# Autodesk Inventor assembly: board_box
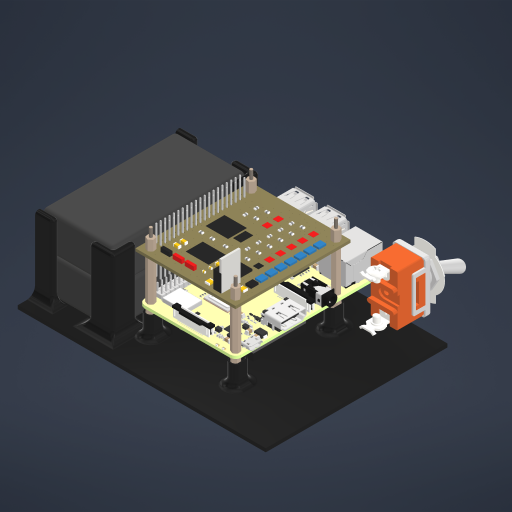
[picture p0: Inventor's stored thumbnail of the model, 512x512]
Saved by Autodesk Inventor 2023 (Build 270158030, 158C)
## iProperties
Created: 2022-07-10
Part Number: board_box
Document SubType Name: Assembly
Designer: Norbert Ligas
Author: Norbert Ligas
## Documents named in this file (10)
- C:\Users\norbe\Repozytoria\NormalMapScanner\3D_modeling\construction\parts\board_box.iam
- C:\Users\norbe\Repozytoria\NormalMapScanner\3D_modeling\power_supply_pcb\power_supply.iam
- C:\Users\norbe\Repozytoria\NormalMapScanner\3D_modeling\construction\parts\board_box\spacer25.ipt
- C:\Users\norbe\Repozytoria\NormalMapScanner\3D_modeling\construction\parts\external_parts\raspberry_pi_3_b_plus\raspberry_pi_3_b_plus.iam
- C:\Users\norbe\Repozytoria\NormalMapScanner\3D_modeling\construction\parts\board_box\RaspberryCameraV2InCase.iam
- C:\Users\norbe\Repozytoria\NormalMapScanner\3D_modeling\construction\parts\board_box\board_box_bottom.ipt
- C:\Users\norbe\Repozytoria\NormalMapScanner\3D_modeling\construction\parts\board_box\RaspberryCameraV2Case.ipt
- C:\Users\norbe\Repozytoria\NormalMapScanner\3D_modeling\construction\parts\board_box\accumulators_case.ipt
- C:\Users\norbe\Repozytoria\NormalMapScanner\3D_modeling\construction\parts\board_box\spacer6.ipt
- C:\Users\norbe\Repozytoria\NormalMapScanner\3D_modeling\construction\parts\board_box\Switch\Switch.iam
## Components (19 placed, 8 different names)
1. raspberry_pi_3_b_plus:2 [sub-assembly] — Mate:20, Mate:22, Mate:34, Mate:35, Mate:36, Mate:42, Mate:46, Mate:47, Mate:54, Mate:55, Mate:56, Mate:58, Mate:60, Mate:62
2. power_supply:1 [sub-assembly] — Mate:41, Mate:44, Mate:45, Mate:63, Mate:65, Mate:66, Mate:67, Mate:68, Mate:69, Mate:71, Mate:73, Mate:75
3. spacer25:1 — Mate:20, Mate:38, Mate:54, Mate:59, Mate:60, Mate:67
4. spacer25:2 — Mate:61, Mate:62, Mate:69, Mate:70
5. spacer25:3 — Mate:22, Mate:63, Mate:65, Mate:66, Mate:72
6. spacer25:4 — Mate:57, Mate:58, Mate:68, Mate:74
7. RaspberryCameraV2InCase:1 [sub-assembly] — Mate:51, Mate:52, Flush:5, Flush:6, Mate:81, Mate:82, Mate:83
8. board_box_bottom:1 — Mate:51, Mate:76, Mate:77, Mate:78, Mate:79, Mate:80, Flush:6, Mate:82, Mate:83, Flush:8, Mate:84, Mate:85, Mate:86
9. accumulators_case:1 — Mate:28, Flush:3, Flush:4, Mate:84, Mate:85, Mate:86
10. accumulators_case:2 — Mate:28, Flush:3, Flush:4
11. spacer6:1 — Mate:55, Mate:56, Mate:57, Mate:76, Mate:79
12. spacer6:2 — Mate:34, Mate:46, Mate:61, Mate:77, Mate:78
13. spacer6:3 — Mate:45, Mate:74, Mate:75
14. spacer6:4 — Mate:72, Mate:73
15. spacer6:5 — Mate:41, Mate:70, Mate:71
16. spacer6:6 — Mate:38, Mate:44
17. spacer6:7 — Mate:36, Mate:47
18. spacer6:8 — Mate:35, Mate:42, Mate:59, Mate:80
19. Switch:1 [sub-assembly] — Flush:8
## Relationships (52: Mate 47, Flush 5)
- Mate:20: raspberry_pi_3_b_plus:2 ↔ spacer25:1
- Mate:22: raspberry_pi_3_b_plus:2 ↔ spacer25:3
- Mate:28: accumulators_case:1 ↔ accumulators_case:2
- Flush:3: accumulators_case:1 ↔ accumulators_case:2
- Flush:4: accumulators_case:1 ↔ accumulators_case:2
- Mate:34: raspberry_pi_3_b_plus:2 ↔ spacer6:2
- Mate:35: raspberry_pi_3_b_plus:2 ↔ spacer6:8
- Mate:36: raspberry_pi_3_b_plus:2 ↔ spacer6:7
- Mate:38: spacer25:1 ↔ spacer6:6
- Mate:41: power_supply:1 ↔ spacer6:5
- Mate:42: raspberry_pi_3_b_plus:2 ↔ spacer6:8
- Mate:44: power_supply:1 ↔ spacer6:6
- Mate:45: power_supply:1 ↔ spacer6:3
- Mate:46: raspberry_pi_3_b_plus:2 ↔ spacer6:2
- Mate:47: raspberry_pi_3_b_plus:2 ↔ spacer6:7
- Mate:51: RaspberryCameraV2InCase:1 ↔ board_box_bottom:1
- Mate:52: RaspberryCameraV2InCase:1
- Mate:54: raspberry_pi_3_b_plus:2 ↔ spacer25:1
- Mate:55: raspberry_pi_3_b_plus:2 ↔ spacer6:1
- Mate:56: raspberry_pi_3_b_plus:2 ↔ spacer6:1
- Mate:57: spacer25:4 ↔ spacer6:1
- Mate:58: raspberry_pi_3_b_plus:2 ↔ spacer25:4
- Mate:59: spacer25:1 ↔ spacer6:8
- Mate:60: raspberry_pi_3_b_plus:2 ↔ spacer25:1
- Mate:61: spacer25:2 ↔ spacer6:2
- Mate:62: raspberry_pi_3_b_plus:2 ↔ spacer25:2
- Mate:63: power_supply:1 ↔ spacer25:3
- Mate:65: power_supply:1 ↔ spacer25:3
- Mate:66: power_supply:1 ↔ spacer25:3
- Mate:67: power_supply:1 ↔ spacer25:1
- Mate:68: power_supply:1 ↔ spacer25:4
- Mate:69: power_supply:1 ↔ spacer25:2
- Mate:70: spacer25:2 ↔ spacer6:5
- Mate:71: power_supply:1 ↔ spacer6:5
- Mate:72: spacer25:3 ↔ spacer6:4
- Mate:73: power_supply:1 ↔ spacer6:4
- Mate:74: spacer25:4 ↔ spacer6:3
- Mate:75: power_supply:1 ↔ spacer6:3
- Mate:76: board_box_bottom:1 ↔ spacer6:1
- Mate:77: board_box_bottom:1 ↔ spacer6:2
- Mate:78: board_box_bottom:1 ↔ spacer6:2
- Mate:79: board_box_bottom:1 ↔ spacer6:1
- Mate:80: board_box_bottom:1 ↔ spacer6:8
- Flush:5: RaspberryCameraV2InCase:1
- Flush:6: RaspberryCameraV2InCase:1 ↔ board_box_bottom:1
- Mate:81: RaspberryCameraV2InCase:1
- Mate:82: RaspberryCameraV2InCase:1 ↔ board_box_bottom:1
- Mate:83: RaspberryCameraV2InCase:1 ↔ board_box_bottom:1
- Flush:8: board_box_bottom:1 ↔ Switch:1
- Mate:84: board_box_bottom:1 ↔ accumulators_case:1
- Mate:85: board_box_bottom:1 ↔ accumulators_case:1
- Mate:86: board_box_bottom:1 ↔ accumulators_case:1
## Named parameters: bottom_rasp_holder_radius_difference = 1 mm, width = 30.5 mm, length = 49.3 mm, opening_width = 3 mm, opening_length = 23.2 mm, opening_distance_to_edge = 3.3 mm, camera_box_width = 30.5 mm, thickness = 3 mm, inside_width = 26.2 mm, height = 12.3 mm, raspberry_pcb_length = 1 mm, raspberry_pcb_width = 1 mm, power_supply_width = 57.8 mm, power_supply_length = 66.4 mm, board_box_inside_width = 1 mm, board_box_inside_length = 1 mm, batteries_case_width = 41 mm, batteries_case_length = 77 mm, batteries_case_height = 21 mm
